# Autodesk Inventor assembly: head
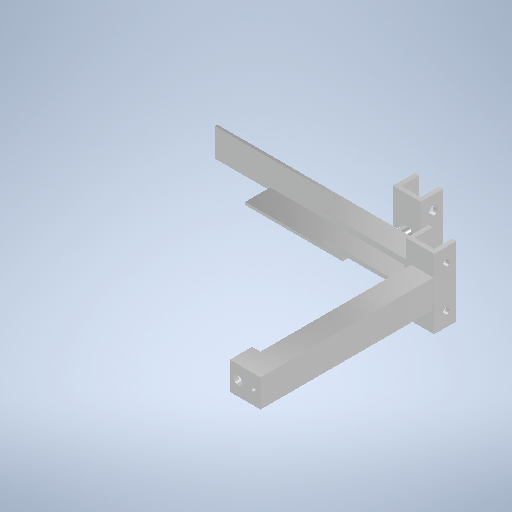
[picture p0: Inventor's stored thumbnail of the model, 512x512]
Saved by Autodesk Inventor 2025 (Build 290162000, 162)
## iProperties
Created: 2024-04-25
Part Number: head
Document SubType Name: Assembly
Designer: rader
Author: rader
## Documents named in this file (7)
- C:\Users\rader\Documents\rp\head.iam
- C:\Users\rader\Documents\rp\x_bearing_holder.ipt
- C:\Users\rader\Documents\rp\head_arm.ipt
- C:\Users\rader\Documents\rp\lift_tab_bracket.ipt
- C:\Users\rader\Documents\rp\standoff.ipt
- C:\Users\rader\Documents\rp\x_belt_anchor.ipt
- C:\Users\rader\Documents\rp\lift_tab.ipt
## Components (6 placed, 6 different names)
1. x_bearing_holder:1 — Proti sobě:1, Vložit:1, Vložit:2
2. head_arm:1 — Vložit:1
3. lift_tab_bracket:1 — Vložit:2, Vložit:3, Vložit:5, Proti sobě:2
4. standoff:1 — Vložit:3, Vložit:4
5. x_belt_anchor:1 — Vložit:4
6. lift_tab:1 — Vložit:5, Proti sobě:2
## Relationships (7: Insert 5, Mate 2)
- Proti sobě:1 [Mate]: x_bearing_holder:1
- Vložit:1 [Insert]: x_bearing_holder:1 ↔ head_arm:1
- Vložit:2 [Insert]: x_bearing_holder:1 ↔ lift_tab_bracket:1
- Vložit:3 [Insert]: lift_tab_bracket:1 ↔ standoff:1
- Vložit:4 [Insert]: standoff:1 ↔ x_belt_anchor:1
- Vložit:5 [Insert]: lift_tab_bracket:1 ↔ lift_tab:1
- Proti sobě:2 [Mate]: lift_tab_bracket:1 ↔ lift_tab:1
